# Autodesk Inventor assembly: 000.005.005 - Сгиб кисти
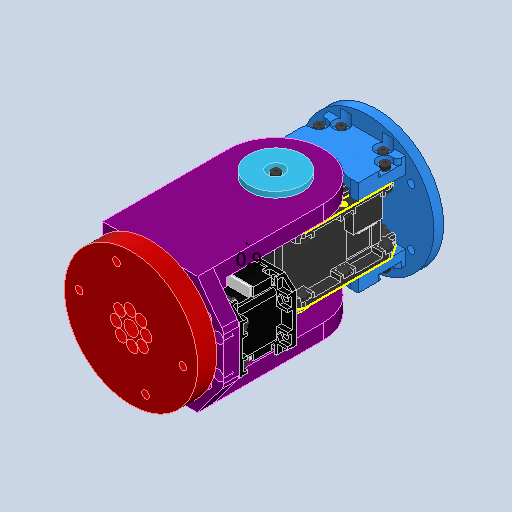
[picture p0: Inventor's stored thumbnail of the model, 512x512]
Saved by Autodesk Inventor 2022 (Build 260153000, 153)
## iProperties
Created: 2022-12-19
Part Number: 000.005.005 - Сгиб кисти
Document SubType Name: Assembly
Designer: Ivan Petrov
Author: Ivan Petrov
## Documents named in this file (15)
- C:\Users\Ivan Petrov\Documents\GitHub\OmniBot\design\000.005.005 - Сгиб кисти.iam
- 000.005.005 - Сгиб кисти СБ.iam
- C:\Users\Ivan Petrov\Documents\GitHub\OmniBot\design\000.005.005.001 - Основание.ipt
- C:\Users\Ivan Petrov\Documents\GitHub\OmniBot\design\standart_components\dynamixels\mx-64\MX-64T.iam
- C:\Users\Ivan Petrov\Documents\GitHub\OmniBot\design\000.005.005.002 - Качалка.ipt
- C:\Users\Ivan Petrov\Documents\GitHub\OmniBot\design\Content Center Files\R2022\ru-RU\SKF 2RS1 -  with two seals\SKF 2RS1608-2RS1.ipt
- C:\Users\Ivan Petrov\Documents\GitHub\OmniBot\design\000.005.005.003 - Втулка.ipt
- C:\Users\Ivan Petrov\Documents\GitHub\OmniBot\design\Content Center Files\ru-RU\DIN 912\DIN 912 - M2,5 x 0,45 x 12 x 10,875.ipt
- C:\Users\Ivan Petrov\Documents\GitHub\OmniBot\design\Content Center Files\ru-RU\AS 1112 (2)\AS 1112 - M2,5  Тип 5.ipt
- C:\Users\Ivan Petrov\Documents\GitHub\OmniBot\design\Content Center Files\ru-RU\DIN 912\DIN 912 - M2,5 x 0,45 x 8 x 6,875.ipt
- C:\Users\Ivan Petrov\Documents\GitHub\OmniBot\design\standart_components\dynamixels\mx-28\MX-28.iam
- C:\Users\Ivan Petrov\Documents\GitHub\OmniBot\design\Content Center Files\ru-RU\DIN 912\DIN 912 - M2,5 x 0,45 x 10 x 8,875.ipt
- C:\Users\Ivan Petrov\Documents\GitHub\OmniBot\design\000.005.005.004 - Поворотный диск.ipt
- C:\Users\Ivan Petrov\Documents\GitHub\OmniBot\design\Content Center Files\ru-RU\DIN 912\DIN 912 - M2 x 0,4 x 6 x 5.ipt
- C:\Users\Ivan Petrov\Documents\GitHub\OmniBot\design\Content Center Files\ru-RU\DIN 912\DIN 912 - M2 x 0,4 x 10 x 9.ipt
## Components (64 placed, 13 different names)
1. 000.005.005.001 - Основание:1 — Совмещение:1, Совмещение:2, Вставка:1, Вставка:2, Вставка:3, Вставка:4, Вставка:5, Вставка:6, Вставка:7, Вставка:8
2. MX-64T:1 [sub-assembly] — Совмещение:1, Совмещение:2, Угол:1, Совмещение:3, Совмещение:4, Совмещение:5, Совмещение:7, Вставка:9, Вставка:10, Вставка:11, Вставка:12, Вставка:13, Вставка:14, Вставка:15, Вставка:16, Вставка:17, Вставка:18, Вставка:19, Вставка:20, Вставка:21, Вставка:22, Вставка:23, Вставка:24, Совмещение:9
3. 000.005.005.003 - Втулка:1 — Совмещение:7, Совмещение:8, Вставка:33
4. MX-28:1 [sub-assembly] — Заподлицо:1, Совмещение:10, Угол:3, Вставка:42, Вставка:43, Вставка:44, Вставка:45, Вставка:46, Вставка:47, Вставка:48, Вставка:49, Совмещение:11, Совмещение:12, Совмещение:13
5. 000.005.005.004 - Поворотный диск:1 — Совмещение:11, Совмещение:12, Вставка:50, Вставка:51, Вставка:52, Вставка:53, Вставка:54, Вставка:55, Вставка:56, Вставка:57, Совмещение:13
6. 000.005.005.002 - Качалка:1 — Совмещение:3, Совмещение:4, Совмещение:6, Совмещение:8, Вставка:25, Вставка:26, Вставка:27, Вставка:28, Вставка:29, Вставка:30, Вставка:31, Вставка:32, Заподлицо:1, Совмещение:10, Угол:3, Вставка:34, Вставка:35, Вставка:36, Вставка:37, Вставка:38, Вставка:39, Вставка:40, Вставка:41
7. DIN 912 - заменено на DIN EN ISO 4762 M2 x 6:1 — Вставка:50
8. DIN 912 - заменено на DIN EN ISO 4762 M2 x 6:2 — Вставка:51
9. DIN 912 - заменено на DIN EN ISO 4762 M2 x 6:3 — Вставка:52
10. DIN 912 - заменено на DIN EN ISO 4762 M2 x 6:4 — Вставка:53
11. DIN 912 - заменено на DIN EN ISO 4762 M2 x 6:5 — Вставка:54
12. DIN 912 - заменено на DIN EN ISO 4762 M2 x 6:6 — Вставка:55
13. DIN 912 - заменено на DIN EN ISO 4762 M2 x 10:1 — Вставка:56
14. DIN 912 - заменено на DIN EN ISO 4762 M2 x 6:8 — Вставка:57
15. DIN 912 - заменено на DIN EN ISO 4762 M2,5 x 10:1 — Вставка:34
16. DIN 912 - заменено на DIN EN ISO 4762 M2,5 x 10:2 — Вставка:35
17. DIN 912 - заменено на DIN EN ISO 4762 M2,5 x 10:3 — Вставка:36
18. DIN 912 - заменено на DIN EN ISO 4762 M2,5 x 10:4 — Вставка:37
19. DIN 912 - заменено на DIN EN ISO 4762 M2,5 x 10:5 — Вставка:38
20. DIN 912 - заменено на DIN EN ISO 4762 M2,5 x 10:6 — Вставка:39
21. DIN 912 - заменено на DIN EN ISO 4762 M2,5 x 10:7 — Вставка:40
22. DIN 912 - заменено на DIN EN ISO 4762 M2,5 x 10:8 — Вставка:41
23. AS 1112 (2) - метрическая M2,5  Тип 5:17 — Вставка:42
24. AS 1112 (2) - метрическая M2,5  Тип 5:18 — Вставка:43
25. AS 1112 (2) - метрическая M2,5  Тип 5:19 — Вставка:44
26. AS 1112 (2) - метрическая M2,5  Тип 5:20 — Вставка:45
27. AS 1112 (2) - метрическая M2,5  Тип 5:21 — Вставка:46
28. AS 1112 (2) - метрическая M2,5  Тип 5:22 — Вставка:47
29. AS 1112 (2) - метрическая M2,5  Тип 5:23 — Вставка:48
30. AS 1112 (2) - метрическая M2,5  Тип 5:24 — Вставка:49
31. DIN 912 - заменено на DIN EN ISO 4762 M2,5 x 12:9 — Вставка:33
32. DIN 912 - заменено на DIN EN ISO 4762 M2,5 x 12:1 — Вставка:1
33. DIN 912 - заменено на DIN EN ISO 4762 M2,5 x 12:2 — Вставка:2
34. DIN 912 - заменено на DIN EN ISO 4762 M2,5 x 12:3 — Вставка:3
35. DIN 912 - заменено на DIN EN ISO 4762 M2,5 x 12:4 — Вставка:4
36. DIN 912 - заменено на DIN EN ISO 4762 M2,5 x 12:5 — Вставка:5
37. DIN 912 - заменено на DIN EN ISO 4762 M2,5 x 12:6 — Вставка:6
38. DIN 912 - заменено на DIN EN ISO 4762 M2,5 x 12:7 — Вставка:7
39. DIN 912 - заменено на DIN EN ISO 4762 M2,5 x 12:8 — Вставка:8
40. AS 1112 (2) - метрическая M2,5  Тип 5:1 — Вставка:9
41. AS 1112 (2) - метрическая M2,5  Тип 5:2 — Вставка:10
42. AS 1112 (2) - метрическая M2,5  Тип 5:3 — Вставка:11
43. AS 1112 (2) - метрическая M2,5  Тип 5:4 — Вставка:12
44. AS 1112 (2) - метрическая M2,5  Тип 5:5 — Вставка:13
45. AS 1112 (2) - метрическая M2,5  Тип 5:6 — Вставка:14
46. AS 1112 (2) - метрическая M2,5  Тип 5:7 — Вставка:15
47. AS 1112 (2) - метрическая M2,5  Тип 5:8 — Вставка:16
48. AS 1112 (2) - метрическая M2,5  Тип 5:9 — Вставка:17
49. AS 1112 (2) - метрическая M2,5  Тип 5:10 — Вставка:18
50. AS 1112 (2) - метрическая M2,5  Тип 5:11 — Вставка:19
51. AS 1112 (2) - метрическая M2,5  Тип 5:12 — Вставка:20
52. AS 1112 (2) - метрическая M2,5  Тип 5:13 — Вставка:21
53. AS 1112 (2) - метрическая M2,5  Тип 5:14 — Вставка:22
54. AS 1112 (2) - метрическая M2,5  Тип 5:15 — Вставка:23
55. AS 1112 (2) - метрическая M2,5  Тип 5:16 — Вставка:24
56. DIN 912 - заменено на DIN EN ISO 4762 M2,5 x 8:1 — Вставка:25
57. DIN 912 - заменено на DIN EN ISO 4762 M2,5 x 8:2 — Вставка:26, Совмещение:9
58. DIN 912 - заменено на DIN EN ISO 4762 M2,5 x 8:3 — Вставка:27
59. DIN 912 - заменено на DIN EN ISO 4762 M2,5 x 8:4 — Вставка:28
60. DIN 912 - заменено на DIN EN ISO 4762 M2,5 x 8:5 — Вставка:29
61. DIN 912 - заменено на DIN EN ISO 4762 M2,5 x 8:6 — Вставка:30
62. DIN 912 - заменено на DIN EN ISO 4762 M2,5 x 8:7 — Вставка:31
63. DIN 912 - заменено на DIN EN ISO 4762 M2,5 x 8:8 — Вставка:32
64. SKF 2RS1, с двумя уплотнениями SKF 2RS1608-2RS1:1 — Совмещение:5, Совмещение:6
## Relationships (73: Insert 57, Mate 13, Angle 2, Flush 1)
- Совмещение:1 [Mate]: 000.005.005.001 - Основание:1 ↔ MX-64T:1
- Совмещение:2 [Mate]: 000.005.005.001 - Основание:1 ↔ MX-64T:1
- Угол:1 [Angle] (0 deg): MX-64T:1
- Совмещение:3 [Mate]: MX-64T:1 ↔ 000.005.005.002 - Качалка:1
- Совмещение:4 [Mate]: MX-64T:1 ↔ 000.005.005.002 - Качалка:1
- Совмещение:5 [Mate] (0.5 mm): MX-64T:1 ↔ SKF 2RS1, с двумя уплотнениями SKF 2RS1608-2RS1:1
- Совмещение:6 [Mate]: 000.005.005.002 - Качалка:1 ↔ SKF 2RS1, с двумя уплотнениями SKF 2RS1608-2RS1:1
- Совмещение:7 [Mate]: MX-64T:1 ↔ 000.005.005.003 - Втулка:1
- Совмещение:8 [Mate]: 000.005.005.003 - Втулка:1 ↔ 000.005.005.002 - Качалка:1
- Вставка:1 [Insert]: 000.005.005.001 - Основание:1 ↔ DIN 912 - заменено на DIN EN ISO 4762 M2,5 x 12:1
- Вставка:2 [Insert]: 000.005.005.001 - Основание:1 ↔ DIN 912 - заменено на DIN EN ISO 4762 M2,5 x 12:2
- Вставка:3 [Insert]: 000.005.005.001 - Основание:1 ↔ DIN 912 - заменено на DIN EN ISO 4762 M2,5 x 12:3
- Вставка:4 [Insert]: 000.005.005.001 - Основание:1 ↔ DIN 912 - заменено на DIN EN ISO 4762 M2,5 x 12:4
- Вставка:5 [Insert]: 000.005.005.001 - Основание:1 ↔ DIN 912 - заменено на DIN EN ISO 4762 M2,5 x 12:5
- Вставка:6 [Insert]: 000.005.005.001 - Основание:1 ↔ DIN 912 - заменено на DIN EN ISO 4762 M2,5 x 12:6
- Вставка:7 [Insert]: 000.005.005.001 - Основание:1 ↔ DIN 912 - заменено на DIN EN ISO 4762 M2,5 x 12:7
- Вставка:8 [Insert]: 000.005.005.001 - Основание:1 ↔ DIN 912 - заменено на DIN EN ISO 4762 M2,5 x 12:8
- Вставка:9 [Insert]: MX-64T:1 ↔ AS 1112 (2) - метрическая M2,5  Тип 5:1
- Вставка:10 [Insert]: MX-64T:1 ↔ AS 1112 (2) - метрическая M2,5  Тип 5:2
- Вставка:11 [Insert]: MX-64T:1 ↔ AS 1112 (2) - метрическая M2,5  Тип 5:3
- Вставка:12 [Insert]: MX-64T:1 ↔ AS 1112 (2) - метрическая M2,5  Тип 5:4
- Вставка:13 [Insert]: MX-64T:1 ↔ AS 1112 (2) - метрическая M2,5  Тип 5:5
- Вставка:14 [Insert]: MX-64T:1 ↔ AS 1112 (2) - метрическая M2,5  Тип 5:6
- Вставка:15 [Insert]: MX-64T:1 ↔ AS 1112 (2) - метрическая M2,5  Тип 5:7
- Вставка:16 [Insert]: MX-64T:1 ↔ AS 1112 (2) - метрическая M2,5  Тип 5:8
- Вставка:17 [Insert]: MX-64T:1 ↔ AS 1112 (2) - метрическая M2,5  Тип 5:9
- Вставка:18 [Insert]: MX-64T:1 ↔ AS 1112 (2) - метрическая M2,5  Тип 5:10
- Вставка:19 [Insert]: MX-64T:1 ↔ AS 1112 (2) - метрическая M2,5  Тип 5:11
- Вставка:20 [Insert]: MX-64T:1 ↔ AS 1112 (2) - метрическая M2,5  Тип 5:12
- Вставка:21 [Insert]: MX-64T:1 ↔ AS 1112 (2) - метрическая M2,5  Тип 5:13
- Вставка:22 [Insert]: MX-64T:1 ↔ AS 1112 (2) - метрическая M2,5  Тип 5:14
- Вставка:23 [Insert]: MX-64T:1 ↔ AS 1112 (2) - метрическая M2,5  Тип 5:15
- Вставка:24 [Insert]: MX-64T:1 ↔ AS 1112 (2) - метрическая M2,5  Тип 5:16
- Вставка:25 [Insert]: 000.005.005.002 - Качалка:1 ↔ DIN 912 - заменено на DIN EN ISO 4762 M2,5 x 8:1
- Вставка:26 [Insert]: 000.005.005.002 - Качалка:1 ↔ DIN 912 - заменено на DIN EN ISO 4762 M2,5 x 8:2
- Вставка:27 [Insert]: 000.005.005.002 - Качалка:1 ↔ DIN 912 - заменено на DIN EN ISO 4762 M2,5 x 8:3
- Вставка:28 [Insert]: 000.005.005.002 - Качалка:1 ↔ DIN 912 - заменено на DIN EN ISO 4762 M2,5 x 8:4
- Вставка:29 [Insert]: 000.005.005.002 - Качалка:1 ↔ DIN 912 - заменено на DIN EN ISO 4762 M2,5 x 8:5
- Вставка:30 [Insert]: 000.005.005.002 - Качалка:1 ↔ DIN 912 - заменено на DIN EN ISO 4762 M2,5 x 8:6
- Вставка:31 [Insert]: 000.005.005.002 - Качалка:1 ↔ DIN 912 - заменено на DIN EN ISO 4762 M2,5 x 8:7
- Вставка:32 [Insert]: 000.005.005.002 - Качалка:1 ↔ DIN 912 - заменено на DIN EN ISO 4762 M2,5 x 8:8
- Совмещение:9 [Mate]: MX-64T:1 ↔ DIN 912 - заменено на DIN EN ISO 4762 M2,5 x 8:2
- Вставка:33 [Insert]: 000.005.005.003 - Втулка:1 ↔ DIN 912 - заменено на DIN EN ISO 4762 M2,5 x 12:9
- Заподлицо:1 [Flush]: MX-28:1 ↔ 000.005.005.002 - Качалка:1
- Совмещение:10 [Mate]: MX-28:1 ↔ 000.005.005.002 - Качалка:1
- Угол:3 [Angle] (0 deg): MX-28:1 ↔ 000.005.005.002 - Качалка:1
- Вставка:34 [Insert]: 000.005.005.002 - Качалка:1 ↔ DIN 912 - заменено на DIN EN ISO 4762 M2,5 x 10:1
- Вставка:35 [Insert]: 000.005.005.002 - Качалка:1 ↔ DIN 912 - заменено на DIN EN ISO 4762 M2,5 x 10:2
- Вставка:36 [Insert]: 000.005.005.002 - Качалка:1 ↔ DIN 912 - заменено на DIN EN ISO 4762 M2,5 x 10:3
- Вставка:37 [Insert]: 000.005.005.002 - Качалка:1 ↔ DIN 912 - заменено на DIN EN ISO 4762 M2,5 x 10:4
- Вставка:38 [Insert]: 000.005.005.002 - Качалка:1 ↔ DIN 912 - заменено на DIN EN ISO 4762 M2,5 x 10:5
- Вставка:39 [Insert]: 000.005.005.002 - Качалка:1 ↔ DIN 912 - заменено на DIN EN ISO 4762 M2,5 x 10:6
- Вставка:40 [Insert]: 000.005.005.002 - Качалка:1 ↔ DIN 912 - заменено на DIN EN ISO 4762 M2,5 x 10:7
- Вставка:41 [Insert]: 000.005.005.002 - Качалка:1 ↔ DIN 912 - заменено на DIN EN ISO 4762 M2,5 x 10:8
- Вставка:42 [Insert]: MX-28:1 ↔ AS 1112 (2) - метрическая M2,5  Тип 5:17
- Вставка:43 [Insert]: MX-28:1 ↔ AS 1112 (2) - метрическая M2,5  Тип 5:18
- Вставка:44 [Insert]: MX-28:1 ↔ AS 1112 (2) - метрическая M2,5  Тип 5:19
- Вставка:45 [Insert]: MX-28:1 ↔ AS 1112 (2) - метрическая M2,5  Тип 5:20
- Вставка:46 [Insert]: MX-28:1 ↔ AS 1112 (2) - метрическая M2,5  Тип 5:21
- Вставка:47 [Insert]: MX-28:1 ↔ AS 1112 (2) - метрическая M2,5  Тип 5:22
- Вставка:48 [Insert]: MX-28:1 ↔ AS 1112 (2) - метрическая M2,5  Тип 5:23
- Вставка:49 [Insert]: MX-28:1 ↔ AS 1112 (2) - метрическая M2,5  Тип 5:24
- Совмещение:11 [Mate]: MX-28:1 ↔ 000.005.005.004 - Поворотный диск:1
- Совмещение:12 [Mate]: MX-28:1 ↔ 000.005.005.004 - Поворотный диск:1
- Вставка:50 [Insert]: 000.005.005.004 - Поворотный диск:1 ↔ DIN 912 - заменено на DIN EN ISO 4762 M2 x 6:1
- Вставка:51 [Insert]: 000.005.005.004 - Поворотный диск:1 ↔ DIN 912 - заменено на DIN EN ISO 4762 M2 x 6:2
- Вставка:52 [Insert]: 000.005.005.004 - Поворотный диск:1 ↔ DIN 912 - заменено на DIN EN ISO 4762 M2 x 6:3
- Вставка:53 [Insert]: 000.005.005.004 - Поворотный диск:1 ↔ DIN 912 - заменено на DIN EN ISO 4762 M2 x 6:4
- Вставка:54 [Insert]: 000.005.005.004 - Поворотный диск:1 ↔ DIN 912 - заменено на DIN EN ISO 4762 M2 x 6:5
- Вставка:55 [Insert]: 000.005.005.004 - Поворотный диск:1 ↔ DIN 912 - заменено на DIN EN ISO 4762 M2 x 6:6
- Вставка:56 [Insert]: 000.005.005.004 - Поворотный диск:1 ↔ DIN 912 - заменено на DIN EN ISO 4762 M2 x 10:1
- Вставка:57 [Insert]: 000.005.005.004 - Поворотный диск:1 ↔ DIN 912 - заменено на DIN EN ISO 4762 M2 x 6:8
- Совмещение:13 [Mate]: MX-28:1 ↔ 000.005.005.004 - Поворотный диск:1
